# Autodesk Inventor assembly: Fidget_Assembly
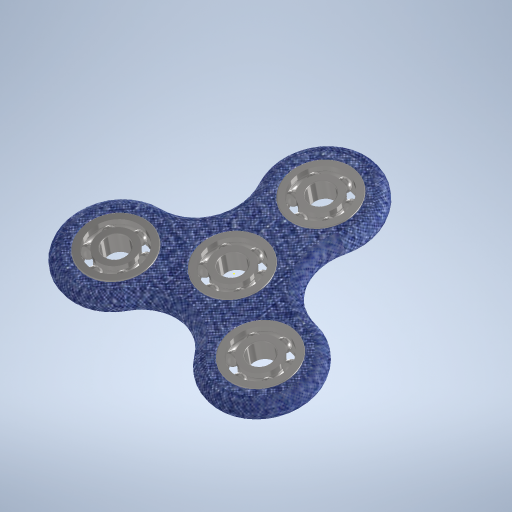
[picture p0: Inventor's stored thumbnail of the model, 512x512]
Saved by Autodesk Inventor 2023 (Build 270158000, 158)
## iProperties
Created: 2023-02-10
Part Number: Fidget_Assembly
Document SubType Name: Assembly
Designer: General
Author: General
## Documents named in this file (4)
- A:\DevOps\Invprojects\exercises\Completed Exercises\FidgetSpinner\Fidget_Assembly.iam
- A:\DevOps\Invprojects\exercises\Completed Exercises\FidgetSpinner\mainbody.ipt
- A:\DevOps\Invprojects\exercises\Completed Exercises\FidgetSpinner\Fidget_Assembly\Design Accelerator\Bearing1.iam
- A:\DevOps\Invprojects\exercises\Completed Exercises\FidgetSpinner\Fidget_Assembly\Design Accelerator\Bearing2.iam
## Components (5 placed, 2 different names)
1. mainbody:1 — Mate:1, Mate:2, Mate:3, Mate:4, Angle:1
2. Bearing:1 [sub-assembly] — Mate:1, Mate:2, Mate:5, Mate:6, Flush:1
3. Bearing:2 [sub-assembly] — Mate:3, Mate:4
4. Bearing:3 [sub-assembly]
5. Bearing:4 [sub-assembly]
## Component patterns: (3 elements, first: Bearing:2)
## Relationships (8: Mate 6, Flush 1, Angle 1)
- Mate:1: mainbody:1 ↔ Bearing:1
- Mate:2: mainbody:1 ↔ Bearing:1
- Mate:3: mainbody:1 ↔ Bearing:2
- Mate:4: mainbody:1 ↔ Bearing:2
- Mate:5: Bearing:1
- Mate:6: Bearing:1
- Flush:1: Bearing:1
- Angle:1 (0 deg): mainbody:1
